# Autodesk Inventor assembly: Hand
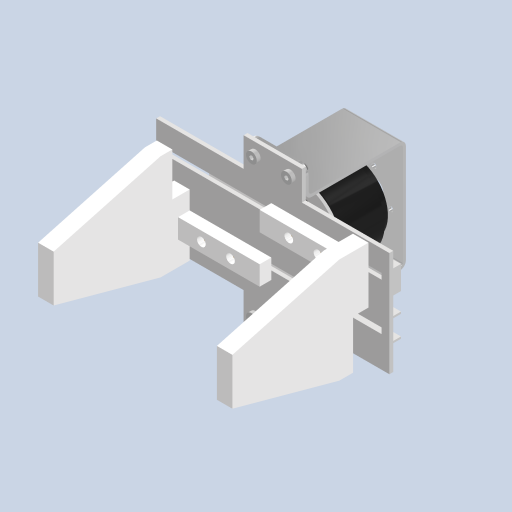
[picture p0: Inventor's stored thumbnail of the model, 512x512]
Saved by Autodesk Inventor 2023 (Build 270158000, 158)
## iProperties
Created: 2024-11-27
Part Number: Hand
Document SubType Name: Assembly
Designer: kiyo
Mass: 142.009 g
Surface Area: 718.919 cm^2
Volume: 132.865 cm^3
Density: 1.06882 g/cm^3
Author: kiyo
## Documents named in this file (13)
- D:\GitHub\inventor\syu-si\OfficeRobot\Hand\Hand.iam
- D:\GitHub\inventor\syu-si\OfficeRobot\ReadyMade\Steadywin\GIM3505-8_with-driver.ipt
- D:\GitHub\inventor\syu-si\OfficeRobot\ReadyMade\Screw\GFM-0304-03.ipt
- D:\GitHub\inventor\syu-si\OfficeRobot\ReadyMade\Screw\FB-305530.ipt
- D:\GitHub\inventor\syu-si\OfficeRobot\ReadyMade\Screw\CBSH3-8.ipt
- D:\GitHub\inventor\syu-si\OfficeRobot\ReadyMade\Screw\M2-5_6mm.ipt
- D:\GitHub\inventor\syu-si\OfficeRobot\Hand\motor-fixing.ipt
- D:\GitHub\inventor\syu-si\OfficeRobot\Hand\hand_box1.ipt
- D:\GitHub\inventor\syu-si\OfficeRobot\Hand\hand_box2.ipt
- D:\GitHub\inventor\syu-si\OfficeRobot\Hand\right-nail.ipt
- D:\GitHub\inventor\syu-si\OfficeRobot\Hand\left-nail.ipt
- D:\GitHub\inventor\syu-si\OfficeRobot\Hand\rackgear.ipt
- D:\GitHub\inventor\syu-si\OfficeRobot\Hand\hand-gear.ipt
## Components (30 placed, 12 different names)
1. GIM3505-8_with-driver:1 — 挿入:45, 挿入:46
2. left-nail:2
3. right-nail:2
4. hand_box1:1 — 挿入:47, 挿入:48, 挿入:53, 挿入:54, 挿入:55, 挿入:56
5. rackgear:4
6. rackgear:3
7. hand-gear
8. motor-fixing:1 — 挿入:45, 挿入:46, 挿入:49, 挿入:50
9. hand_box2:1 — 挿入:47, 挿入:48, 挿入:51, 挿入:52
10. CBSH3-8:1
11. CBSH3-8:2
12. CBSH3-8:3
13. CBSH3-8:4
14. CBSH3-8:5 — 挿入:53
15. CBSH3-8:6 — 挿入:54
16. CBSH3-8:7 — 挿入:55
17. CBSH3-8:8 — 挿入:56
18. M2-5_6mm:1
19. M2-5_6mm:2
20. M2-5_6mm:3
21. FB-305530:5 — 挿入:50, 挿入:52
22. FB-305530:6 — 挿入:49, 挿入:51
23. GFM-0304-03:1
24. GFM-0304-03:2
25. GFM-0304-03:3
26. GFM-0304-03:4
27. FB-305530:1
28. FB-305530:2
29. FB-305530:3
30. FB-305530:4
## Relationships (38: Insert 32, Mate 4, Flush 2)
- [Insert]: GIM3505-8_with-driver:1 ↔ hand-gear
- [Mate] (0.05 mm): hand_box1:1 ↔ rackgear:3
- [Mate] (0.05 mm): hand_box1:1 ↔ rackgear:4
- [Insert]: left-nail:2 ↔ GFM-0304-03:1
- [Insert]: left-nail:2 ↔ GFM-0304-03:2
- [Insert]: rackgear:3 ↔ GFM-0304-03:2
- [Insert]: rackgear:3 ↔ GFM-0304-03:1
- [Mate]: hand_box1:1 ↔ GFM-0304-03:1
- [Insert]: right-nail:2 ↔ GFM-0304-03:3
- [Insert]: right-nail:2 ↔ GFM-0304-03:4
- [Mate]: hand_box1:1 ↔ GFM-0304-03:3
- [Insert]: rackgear:4 ↔ GFM-0304-03:3
- [Insert]: rackgear:4 ↔ GFM-0304-03:4
- [Insert]: right-nail:2 ↔ FB-305530:1
- [Insert]: right-nail:2 ↔ FB-305530:2
- [Insert]: left-nail:2 ↔ FB-305530:4
- [Insert]: left-nail:2 ↔ FB-305530:3
- [Insert]: rackgear:3 ↔ CBSH3-8:4
- [Insert]: rackgear:3 ↔ CBSH3-8:3
- [Insert]: rackgear:4 ↔ CBSH3-8:2
- [Insert]: rackgear:4 ↔ CBSH3-8:1
- [Flush] (60 mm): right-nail:2 ↔ hand_box1:1
- [Flush] (60 mm): left-nail:2 ↔ hand_box1:1
- [Insert]: hand-gear ↔ M2-5_6mm:3
- [Insert]: hand-gear ↔ M2-5_6mm:2
- [Insert]: hand-gear ↔ M2-5_6mm:1
- 挿入:45 [Insert]: GIM3505-8_with-driver:1 ↔ motor-fixing:1
- 挿入:46 [Insert]: GIM3505-8_with-driver:1 ↔ motor-fixing:1
- 挿入:47 [Insert]: hand_box1:1 ↔ hand_box2:1
- 挿入:48 [Insert]: hand_box1:1 ↔ hand_box2:1
- 挿入:49 [Insert]: motor-fixing:1 ↔ FB-305530:6
- 挿入:50 [Insert]: motor-fixing:1 ↔ FB-305530:5
- 挿入:51 [Insert]: hand_box2:1 ↔ FB-305530:6
- 挿入:52 [Insert]: hand_box2:1 ↔ FB-305530:5
- 挿入:53 [Insert]: hand_box1:1 ↔ CBSH3-8:5
- 挿入:54 [Insert]: hand_box1:1 ↔ CBSH3-8:6
- 挿入:55 [Insert]: hand_box1:1 ↔ CBSH3-8:7
- 挿入:56 [Insert]: hand_box1:1 ↔ CBSH3-8:8
